# Autodesk Inventor assembly: Actiu Table with Legs
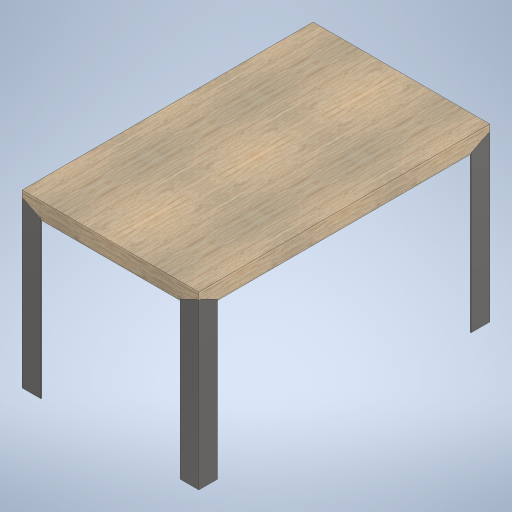
[picture p0: Inventor's stored thumbnail of the model, 512x512]
Saved by Autodesk Inventor 2024 (Build 280153000, 153)
## iProperties
Created: 2021-09-14
Part Number: Actiu Table with Legs
Document SubType Name: Assembly
Designer: sauliusd
Author: sauliusd
## Documents named in this file (3)
- C:\W4INV 2024 Design\PROJECTS\Samples\Macro DEMO\6 Actiu Table\Actiu Table with Legs.iam
- C:\W4INV 2024 Design\PROJECTS\Samples\Macro DEMO\6 Actiu Table\Actiu  Glued TableTop.ipt
- C:\W4INV 2024 Design\PROJECTS\Samples\Macro DEMO\6 Actiu Table\Leg of table.ipt
## Components (5 placed, 2 different names)
1. Actiu  Glued TableTop:1 — Side Plane 2:1, Side Plane 1:1, Bottom Plane:1, Side Plane 1:2, Side Plane 2:2, Bottom Plane:2, Side Plane 1:3, Side Plane 2:3, Bottom Plane:3, Side Plane 1:4, Side Plane 2:4, Bottom Plane:4
2. Leg of table:1 — Side Plane 2:1, Side Plane 1:1, Bottom Plane:1
3. Leg of table:2 — Side Plane 1:2, Side Plane 2:2, Bottom Plane:2
4. Leg of table:3 — Side Plane 1:4, Side Plane 2:4, Bottom Plane:4
5. Leg of table:4 — Side Plane 1:3, Side Plane 2:3, Bottom Plane:3
## Relationships (12: Flush 12)
- Side Plane 2:1 [Flush]: Actiu  Glued TableTop:1 ↔ Leg of table:1
- Side Plane 1:1 [Flush]: Actiu  Glued TableTop:1 ↔ Leg of table:1
- Bottom Plane:1 [Flush]: Actiu  Glued TableTop:1 ↔ Leg of table:1
- Side Plane 1:2 [Flush]: Actiu  Glued TableTop:1 ↔ Leg of table:2
- Side Plane 2:2 [Flush]: Actiu  Glued TableTop:1 ↔ Leg of table:2
- Bottom Plane:2 [Flush]: Actiu  Glued TableTop:1 ↔ Leg of table:2
- Side Plane 1:3 [Flush]: Actiu  Glued TableTop:1 ↔ Leg of table:4
- Side Plane 2:3 [Flush]: Actiu  Glued TableTop:1 ↔ Leg of table:4
- Bottom Plane:3 [Flush]: Actiu  Glued TableTop:1 ↔ Leg of table:4
- Side Plane 1:4 [Flush]: Actiu  Glued TableTop:1 ↔ Leg of table:3
- Side Plane 2:4 [Flush]: Actiu  Glued TableTop:1 ↔ Leg of table:3
- Bottom Plane:4 [Flush]: Actiu  Glued TableTop:1 ↔ Leg of table:3
